# Autodesk Inventor assembly: robo_mdf
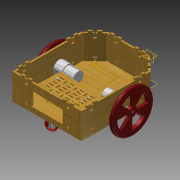
[picture p0: Inventor's stored thumbnail of the model, 180x180]
Saved by Autodesk Inventor 2014 (Build 180170000, 170)
## iProperties
Created: 2014-11-10
Part Number: robo_mdf
Document SubType Name: Assembly
Designer: Gabriel
Author: Gabriel
## Documents named in this file (11)
- C:\Users\Gabriel\Desktop\Esboço_robô\rodabobagrande\robo_mdf.iam
- C:\Users\Gabriel\Desktop\Esboço_robô\rodabobagrande\chassi_mdf.ipt
- C:\Users\Gabriel\Desktop\Esboço_robô\rodabobagrande\lateral_mdf.ipt
- C:\Users\Gabriel\Desktop\Esboço_robô\rodabobagrande\lateral_mdf2.ipt
- C:\Users\Gabriel\Desktop\Esboço_robô\rodabobagrande\frontal.ipt
- C:\Users\Gabriel\Desktop\Esboço_robô\rodabobagrande\motor_polulu.ipt
- C:\Users\Gabriel\Desktop\Esboço_robô\rodabobagrande\parafuso.ipt
- C:\Users\Gabriel\Desktop\Esboço_robô\rodabobagrande\suporte.ipt
- C:\Users\Gabriel\Desktop\Esboço_robô\rodabobagrande\roda_boba.iam
- C:\Users\Gabriel\Desktop\Esboço_robô\rodabobagrande\roda_mdf.ipt
- C:\Users\Gabriel\Desktop\Esboço_robô\rodabobagrande\lateralnova.ipt
## Components (17 placed, 10 different names)
1. chassi_mdf:1 — Cylindrical:1, Cylindrical:19, Cylindrical:18, Cylindrical:17, Rigid:13, Rigid:14, Rigid:15, Rigid:19, Rotational:6, Rigid:24, Rigid:25
2. parafuso:1 — Cylindrical:18
3. parafuso:3 — Cylindrical:19
4. parafuso:4 — Cylindrical:1
5. suporte:1 — Cylindrical:17
6. lateral_mdf:1 — Rigid:13, Rotational:4
7. motor_polulu:1 — Rotational:4, Rotational:5
8. lateral_mdf:2 — Rigid:14, Rigid:21, Rotational:7
9. lateral_mdf2:1 — Rigid:15
10. frontal:1 — Rigid:19
11. roda_mdf:1 — Rotational:5
12. chassi_mdf:2 — Rigid:21
13. roda_boba:1 [sub-assembly] — Rotational:6
14. motor_polulu:2 — Rotational:7, Rigid:22
15. roda_mdf:2 — Rigid:22
16. lateralnova:2 — Rigid:24
17. lateralnova:3 — Rigid:25
## Relationships (16: WeldJoint 8, CylindricalJoint 4, RevoluteJoint 4)
- Cylindrical:1: chassi_mdf:1 ↔ parafuso:4
- Cylindrical:19: chassi_mdf:1 ↔ parafuso:3
- Cylindrical:18: chassi_mdf:1 ↔ parafuso:1
- Cylindrical:17: chassi_mdf:1 ↔ suporte:1
- Rigid:13 [WeldJoint]: chassi_mdf:1 ↔ lateral_mdf:1
- Rotational:4 [RevoluteJoint]: lateral_mdf:1 ↔ motor_polulu:1
- Rigid:14 [WeldJoint]: chassi_mdf:1 ↔ lateral_mdf:2
- Rigid:15 [WeldJoint]: chassi_mdf:1 ↔ lateral_mdf2:1
- Rotational:5 [RevoluteJoint]: motor_polulu:1 ↔ roda_mdf:1
- Rigid:19 [WeldJoint]: chassi_mdf:1 ↔ frontal:1
- Rigid:21 [WeldJoint]: lateral_mdf:2 ↔ chassi_mdf:2
- Rotational:6 [RevoluteJoint]: chassi_mdf:1 ↔ roda_boba:1
- Rotational:7 [RevoluteJoint]: lateral_mdf:2 ↔ motor_polulu:2
- Rigid:22 [WeldJoint]: motor_polulu:2 ↔ roda_mdf:2
- Rigid:24 [WeldJoint]: chassi_mdf:1 ↔ lateralnova:2
- Rigid:25 [WeldJoint]: chassi_mdf:1 ↔ lateralnova:3
